# Autodesk Inventor assembly: Servo Motor
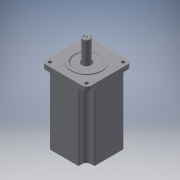
[picture p0: Inventor's stored thumbnail of the model, 180x180]
Saved by Autodesk Inventor 2016 (Build 200138000, 138)
## iProperties
Created: 2017-05-16
Part Number: Servo Motor
Document SubType Name: Assembly
Designer: M220404
Author: M220404
## Documents named in this file (3)
- C:\Users\M220404\Documents\CNC-Lathe-CAD\Servo Motor\Servo Motor.iam
- C:\Users\M220404\Desktop\Part1.ipt
- C:\Users\M220404\Desktop\Part2.ipt
## Components (2 placed, 2 different names)
1. Part1:1 — Mate:1, Mate:2
2. Part2:1 — Mate:1, Mate:2
## Relationships (2: Mate 2)
- Mate:1: Part1:1 ↔ Part2:1
- Mate:2: Part1:1 ↔ Part2:1
